# Autodesk Inventor assembly: gantry_frame
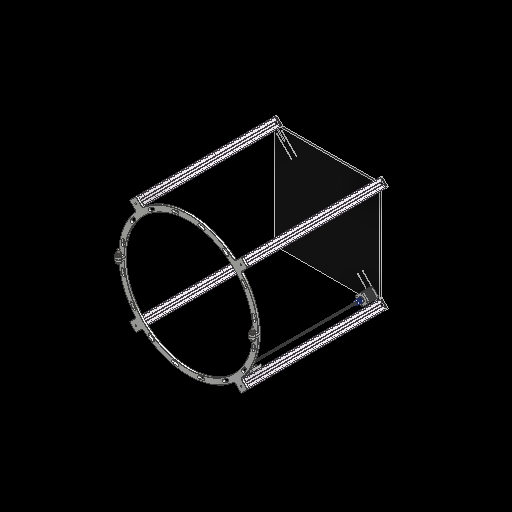
[picture p0: Inventor's stored thumbnail of the model, 512x512]
Saved by Autodesk Inventor 2026.1 (Build 301233000, 233)
## iProperties
Created: 2025-09-18
Part Number: gantry_frame
Document SubType Name: Assembly
Designer: drago
Author: drago
## Documents named in this file (8)
- C:\Users\drago\Desktop\_QIST4500_Multidisciplinary_Team_Project\Proteox MX magnet positioner CAD\gantry_frame.iam
- C:\Users\drago\Desktop\_QIST4500_Multidisciplinary_Team_Project\Proteox MX magnet positioner CAD\half_ring.ipt
- C:\Users\drago\Desktop\_QIST4500_Multidisciplinary_Team_Project\Proteox MX magnet positioner CAD\square_bar.ipt
- C:\Users\drago\Desktop\_QIST4500_Multidisciplinary_Team_Project\Proteox MX magnet positioner CAD\base_plate.ipt
- C:\Users\drago\Documents\Inventor\Content Center Files\R2026\en-US\ISO 7089\ISO 7089 - 10 - 140 HV(1).ipt
- C:\Users\drago\Documents\Inventor\Content Center Files\R2026\en-US\ISO 4014(2)\ISO 4014 - M10 x 45 - ISO.ipt
- C:\Users\drago\Documents\Inventor\Content Center Files\R2026\en-US\ISO 4032(2)\ISO 4032 - M10 - ISO.ipt
- C:\Users\drago\Desktop\_QIST4500_Multidisciplinary_Team_Project\Proteox MX magnet positioner CAD\z_translator\z_Translator.iam
## Components (16 placed, 7 different names)
1. half_ring:1 — Mate:1, Mate:4, Mate:24, Mate:28
2. half_ring:2 — Mate:2, Mate:3, Mate:17, Mate:18, Mate:21, Mate:22, Mate:23, Mate:25, Mate:26, Mate:27
3. base_plate:1 — Mate:19, Angle:8, Mate:31, Mate:32, Mate:33
4. ISO 7089 10:1 — Mate:21, Mate:22, Insert:1
5. ISO 4014 M10 x 45:1 — Insert:1
6. ISO 7089 10:2 — Mate:23, Mate:24, Insert:2
7. ISO 4032 M10:1 — Insert:2
8. ISO 7089 10:3 — Mate:25, Mate:26, Insert:3
9. ISO 4014 M10 x 45:2 — Insert:3
10. ISO 7089 10:4 — Mate:27, Mate:28, Insert:4
11. ISO 4032 M10:2 — Insert:4
12. z_Translator:1 [sub-assembly] — Mate:30, Mate:32, Mate:33
13. square_bar:1 — Mate:17, Angle:7, Mate:18, Mate:30
14. square_bar:2
15. square_bar:3 — Mate:31
16. square_bar:4
## Component patterns: (4 elements, first: square_bar:1)
## Relationships (25: Mate 19, Insert 4, Angle 2)
- Mate:1: half_ring:1
- Mate:2: half_ring:2
- Mate:3: half_ring:2
- Mate:4: half_ring:1
- Mate:17: half_ring:2 ↔ square_bar:1
- Angle:7 (45 deg): square_bar:1
- Mate:18: half_ring:2 ↔ square_bar:1
- Mate:19: base_plate:1
- Angle:8 (45 deg): base_plate:1
- Mate:21: half_ring:2 ↔ ISO 7089 10:1
- Mate:22: half_ring:2 ↔ ISO 7089 10:1
- Insert:1: ISO 7089 10:1 ↔ ISO 4014 M10 x 45:1
- Mate:23: half_ring:2 ↔ ISO 7089 10:2
- Mate:24: half_ring:1 ↔ ISO 7089 10:2
- Insert:2: ISO 7089 10:2 ↔ ISO 4032 M10:1
- Mate:25: half_ring:2 ↔ ISO 7089 10:3
- Mate:26: half_ring:2 ↔ ISO 7089 10:3
- Insert:3: ISO 7089 10:3 ↔ ISO 4014 M10 x 45:2
- Mate:27: half_ring:2 ↔ ISO 7089 10:4
- Mate:28: half_ring:1 ↔ ISO 7089 10:4
- Insert:4: ISO 7089 10:4 ↔ ISO 4032 M10:2
- Mate:30: z_Translator:1 ↔ square_bar:1
- Mate:31: base_plate:1 ↔ square_bar:3
- Mate:32: base_plate:1 ↔ z_Translator:1
- Mate:33: base_plate:1 ↔ z_Translator:1
